# Autodesk Inventor assembly: Knee
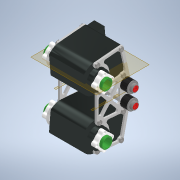
[picture p0: Inventor's stored thumbnail of the model, 180x180]
Saved by Autodesk Inventor 2022.4 (Build 264492000, 492)
## iProperties
Created: 2021-09-07
Part Number: Knee
Document SubType Name: Assembly
Designer: Masato
Mass: 292.217 g
Surface Area: 518.3 cm^2
Volume: 133.122 cm^3
Density: 2.1951 g/cm^3
Author: Masato
## Documents named in this file (16)
- C:\Users\supra\Documents\GitHub\OpenPlatform_ver3_0\LowerBody\Knee\Knee.iam
- C:\Users\supra\Documents\GitHub\OpenPlatform_ver3_0\LowerBody\Knee\Knee_side_frame.ipt
- C:\Users\supra\Documents\GitHub\OpenPlatform_ver3_0\Ready_Made\B3M11xx.ipt
- B3M11xx.ipt
- C:\Users\supra\Documents\GitHub\OpenPlatform_ver3_0\LowerBody\Knee\Knee_clamp.ipt
- C:\Users\supra\Documents\GitHub\OpenPlatform_ver3_0\Ready_Made\FreeHorn.ipt
- C:\Users\supra\Documents\GitHub\OpenPlatform_ver3_0\Ready_Made\SLSBF6-39_5-M3-N3.ipt
- C:\Users\supra\Documents\GitHub\OpenPlatform_ver3_0\Ready_Made\UUW-0312-10BH.ipt
- C:\Users\supra\Documents\GitHub\OpenPlatform_ver3_0\Ready_Made\WSSS-12-10-8.ipt
- C:\Users\supra\Documents\GitHub\OpenPlatform_ver3_0\Ready_Made\BRU-311S.ipt
- C:\Users\supra\Documents\GitHub\OpenPlatform_ver3_0\Ready_Made\80F-0603.ipt
- C:\Users\supra\Documents\GitHub\OpenPlatform_ver3_0\Ready_Made\Screw\M2_6-15.ipt
- C:\Users\supra\Documents\GitHub\OpenPlatform_ver3_0\Ready_Made\Screw\M2_6-20.ipt
- C:\Users\supra\Documents\GitHub\OpenPlatform_ver3_0\Ready_Made\CC-0612-15B.ipt
- C:\Users\supra\Documents\GitHub\OpenPlatform_ver3_0\Ready_Made\CC-0612-50B.ipt
- C:\Users\supra\Documents\GitHub\OpenPlatform_ver3_0\Ready_Made\Screw\FreeHorn_Screw.ipt
## Components (54 placed, 14 different names)
1. Knee_side_frame:1 — 挿入:1, 挿入:2, 挿入:3, 挿入:4, 挿入:5, 挿入:6, 挿入:7, 挿入:8, フラッシュ:4, 挿入:41, 挿入:42, 挿入:45, 挿入:46, 挿入:93, 挿入:94, 挿入:95, 挿入:96, 挿入:97, 挿入:98, 挿入:99, 挿入:100
2. Knee_side_frame:2 — 挿入:9, 挿入:10, 挿入:11, 挿入:12, 挿入:13, 挿入:14, 挿入:15, 挿入:16, 挿入:43, 挿入:44, 挿入:47, 挿入:48, フラッシュ:5, 挿入:85, 挿入:86, 挿入:87, 挿入:88, 挿入:89, 挿入:90, 挿入:91, 挿入:92
3. B3M11xx:1 — 挿入:1, 挿入:2, 挿入:5, 挿入:6, 挿入:9, 挿入:10, 挿入:15, 挿入:16, 挿入:31, 挿入:33, 挿入:112
4. B3M11xx:2 — 挿入:3, 挿入:4, 挿入:7, 挿入:8, 挿入:11, 挿入:12, 挿入:13, 挿入:14, 挿入:32, 挿入:34, 挿入:113
5. Knee_clamp:1 — 挿入:32, 挿入:61
6. Knee_clamp:2 — 挿入:31, 挿入:62
7. Knee_clamp:3 — 挿入:36, 挿入:63
8. Knee_clamp:4 — 挿入:35, 挿入:64
9. FreeHorn:1 — 挿入:33, 挿入:35
10. FreeHorn:2 — 挿入:34, 挿入:36
11. SLSBF6-39_5-M3-N3:1 — 挿入:41, 挿入:43
12. SLSBF6-39_5-M3-N3:2 — 挿入:42, 挿入:44
13. UUW-0312-10BH:1 — 挿入:45, 挿入:77, 挿入:107
14. UUW-0312-10BH:2 — 挿入:46, 挿入:78, 挿入:108
15. UUW-0312-10BH:3 — 挿入:47, 挿入:79, 挿入:106
16. UUW-0312-10BH:4 — 挿入:48, 挿入:80, 挿入:105
17. WSSS-12-10-8:1 — 挿入:64
18. WSSS-12-10-8:2 — 挿入:63
19. WSSS-12-10-8:3 — 挿入:62
20. WSSS-12-10-8:4 — 挿入:61, メイト:1
21. BRU-311S:1 — 挿入:77
22. BRU-311S:2 — 挿入:78
23. BRU-311S:3 — 挿入:80
24. BRU-311S:4 — 挿入:79
25. 80F-0603:1 — 挿入:110
26. 80F-0603:2 — 挿入:109
27. 80F-0603:3 — 挿入:114
28. 80F-0603:4 — 挿入:111
29. M2_6-15:1 — 挿入:85
30. M2_6-15:2 — 挿入:86
31. M2_6-15:3 — 挿入:87
32. M2_6-15:4 — 挿入:88
33. M2_6-15:5 — 挿入:89
34. M2_6-15:6 — 挿入:90
35. M2_6-15:7 — 挿入:91
36. M2_6-15:8 — 挿入:92
37. M2_6-20:1 — 挿入:93
38. M2_6-20:2 — 挿入:94
39. M2_6-20:3 — 挿入:95
40. M2_6-20:4 — 挿入:96
41. M2_6-20:5 — 挿入:97
42. M2_6-20:6 — 挿入:98
43. M2_6-20:7 — 挿入:99
44. M2_6-20:8 — 挿入:100
45. CC-0612-15B:1 — 挿入:101, 挿入:105
46. CC-0612-15B:2 — 挿入:102, 挿入:106
47. CC-0612-15B:3 — 挿入:103, 挿入:107
48. CC-0612-15B:4 — 挿入:104, 挿入:108
49. CC-0612-50B:1 — 挿入:101, 挿入:114
50. CC-0612-50B:2 — 挿入:102, 挿入:111
51. CC-0612-50B:3 — 挿入:103, 挿入:109
52. CC-0612-50B:4 — 挿入:104, 挿入:110
53. FreeHorn_Screw:1 — 挿入:112
54. FreeHorn_Screw:2 — 挿入:113
## Relationships (71: Insert 68, Flush 2, Mate 1)
- 挿入:1 [Insert]: Knee_side_frame:1 ↔ B3M11xx:1
- 挿入:2 [Insert]: Knee_side_frame:1 ↔ B3M11xx:1
- 挿入:3 [Insert]: Knee_side_frame:1 ↔ B3M11xx:2
- 挿入:4 [Insert]: Knee_side_frame:1 ↔ B3M11xx:2
- 挿入:5 [Insert]: Knee_side_frame:1 ↔ B3M11xx:1
- 挿入:6 [Insert]: Knee_side_frame:1 ↔ B3M11xx:1
- 挿入:7 [Insert]: Knee_side_frame:1 ↔ B3M11xx:2
- 挿入:8 [Insert]: Knee_side_frame:1 ↔ B3M11xx:2
- 挿入:9 [Insert]: Knee_side_frame:2 ↔ B3M11xx:1
- 挿入:10 [Insert]: Knee_side_frame:2 ↔ B3M11xx:1
- 挿入:11 [Insert]: Knee_side_frame:2 ↔ B3M11xx:2
- 挿入:12 [Insert]: Knee_side_frame:2 ↔ B3M11xx:2
- 挿入:13 [Insert]: Knee_side_frame:2 ↔ B3M11xx:2
- 挿入:14 [Insert]: Knee_side_frame:2 ↔ B3M11xx:2
- 挿入:15 [Insert]: Knee_side_frame:2 ↔ B3M11xx:1
- 挿入:16 [Insert]: Knee_side_frame:2 ↔ B3M11xx:1
- 挿入:31 [Insert]: B3M11xx:1 ↔ Knee_clamp:2
- 挿入:32 [Insert]: B3M11xx:2 ↔ Knee_clamp:1
- 挿入:33 [Insert]: B3M11xx:1 ↔ FreeHorn:1
- 挿入:34 [Insert]: B3M11xx:2 ↔ FreeHorn:2
- 挿入:35 [Insert]: Knee_clamp:4 ↔ FreeHorn:1
- 挿入:36 [Insert]: Knee_clamp:3 ↔ FreeHorn:2
- フラッシュ:4 [Flush] (-19.75 mm): Knee_side_frame:1
- 挿入:41 [Insert]: Knee_side_frame:1 ↔ SLSBF6-39_5-M3-N3:1
- 挿入:42 [Insert]: Knee_side_frame:1 ↔ SLSBF6-39_5-M3-N3:2
- 挿入:43 [Insert]: Knee_side_frame:2 ↔ SLSBF6-39_5-M3-N3:1
- 挿入:44 [Insert]: Knee_side_frame:2 ↔ SLSBF6-39_5-M3-N3:2
- 挿入:45 [Insert]: Knee_side_frame:1 ↔ UUW-0312-10BH:1
- 挿入:46 [Insert]: Knee_side_frame:1 ↔ UUW-0312-10BH:2
- 挿入:47 [Insert]: Knee_side_frame:2 ↔ UUW-0312-10BH:3
- 挿入:48 [Insert]: Knee_side_frame:2 ↔ UUW-0312-10BH:4
- 挿入:61 [Insert]: Knee_clamp:1 ↔ WSSS-12-10-8:4
- 挿入:62 [Insert]: Knee_clamp:2 ↔ WSSS-12-10-8:3
- 挿入:63 [Insert]: Knee_clamp:3 ↔ WSSS-12-10-8:2
- 挿入:64 [Insert]: Knee_clamp:4 ↔ WSSS-12-10-8:1
- 挿入:77 [Insert]: UUW-0312-10BH:1 ↔ BRU-311S:1
- 挿入:78 [Insert]: UUW-0312-10BH:2 ↔ BRU-311S:2
- 挿入:79 [Insert]: UUW-0312-10BH:3 ↔ BRU-311S:4
- 挿入:80 [Insert]: UUW-0312-10BH:4 ↔ BRU-311S:3
- フラッシュ:5 [Flush]: Knee_side_frame:2
- 挿入:85 [Insert]: Knee_side_frame:2 ↔ M2_6-15:1
- 挿入:86 [Insert]: Knee_side_frame:2 ↔ M2_6-15:2
- 挿入:87 [Insert]: Knee_side_frame:2 ↔ M2_6-15:3
- 挿入:88 [Insert]: Knee_side_frame:2 ↔ M2_6-15:4
- 挿入:89 [Insert]: Knee_side_frame:2 ↔ M2_6-15:5
- 挿入:90 [Insert]: Knee_side_frame:2 ↔ M2_6-15:6
- 挿入:91 [Insert]: Knee_side_frame:2 ↔ M2_6-15:7
- 挿入:92 [Insert]: Knee_side_frame:2 ↔ M2_6-15:8
- 挿入:93 [Insert]: Knee_side_frame:1 ↔ M2_6-20:1
- 挿入:94 [Insert]: Knee_side_frame:1 ↔ M2_6-20:2
- 挿入:95 [Insert]: Knee_side_frame:1 ↔ M2_6-20:3
- 挿入:96 [Insert]: Knee_side_frame:1 ↔ M2_6-20:4
- 挿入:97 [Insert]: Knee_side_frame:1 ↔ M2_6-20:5
- 挿入:98 [Insert]: Knee_side_frame:1 ↔ M2_6-20:6
- 挿入:99 [Insert]: Knee_side_frame:1 ↔ M2_6-20:7
- 挿入:100 [Insert]: Knee_side_frame:1 ↔ M2_6-20:8
- 挿入:101 [Insert]: CC-0612-15B:1 ↔ CC-0612-50B:1
- 挿入:102 [Insert]: CC-0612-15B:2 ↔ CC-0612-50B:2
- 挿入:103 [Insert]: CC-0612-15B:3 ↔ CC-0612-50B:3
- 挿入:104 [Insert]: CC-0612-15B:4 ↔ CC-0612-50B:4
- 挿入:105 [Insert]: UUW-0312-10BH:4 ↔ CC-0612-15B:1
- 挿入:106 [Insert]: UUW-0312-10BH:3 ↔ CC-0612-15B:2
- 挿入:107 [Insert]: UUW-0312-10BH:1 ↔ CC-0612-15B:3
- 挿入:108 [Insert]: UUW-0312-10BH:2 ↔ CC-0612-15B:4
- 挿入:109 [Insert]: 80F-0603:2 ↔ CC-0612-50B:3
- 挿入:110 [Insert]: 80F-0603:1 ↔ CC-0612-50B:4
- 挿入:111 [Insert]: 80F-0603:4 ↔ CC-0612-50B:2
- 挿入:112 [Insert]: B3M11xx:1 ↔ FreeHorn_Screw:1
- 挿入:113 [Insert]: B3M11xx:2 ↔ FreeHorn_Screw:2
- 挿入:114 [Insert]: 80F-0603:3 ↔ CC-0612-50B:1
- メイト:1 [Mate]: WSSS-12-10-8:4
